# Autodesk Inventor assembly: Chain(d)
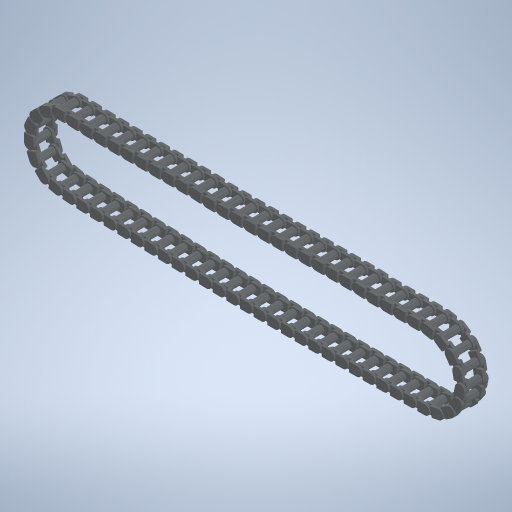
[picture p0: Inventor's stored thumbnail of the model, 512x512]
Saved by Autodesk Inventor 2023 (Build 270158000, 158)
## iProperties
Created: 2022-08-08
Part Number: Chain(d)
Document SubType Name: Assembly
Designer: aaron
Author: aaron
## Documents named in this file (3)
- C:\Users\aaron\Documents\Inventor\Spin Up\library\Motion\New Sprockets\Chain(d).iam
- C:\Users\aaron\Documents\Inventor\Spin Up\library\Motion\New Sprockets\16T.ipt
- C:\Users\aaron\Documents\Inventor\Spin Up\library\Motion\New Sprockets\IQ chain.ipt
## Components (71 placed, 2 different names)
1. 16T:1 — Mate:1, Flush:1, Mate:97, Mate:98, Mate:99, Mate:100, Mate:101, Mate:102, Mate:103, Mate:104, Mate:105
2. 16T:2 — Mate:1, Flush:1, Mate:106, Mate:107, Mate:108, Mate:109, Mate:110, Mate:111, Mate:112, Mate:113, Flush:97
3. IQ chain:6 — Mate:12, Flush:12, Mate:113, Mate:114
4. IQ chain:7 — Mate:12, Flush:12, Mate:112
5. IQ chain:8 — Mate:111
6. IQ chain:9 — Mate:110
7. IQ chain:10 — Mate:109
8. IQ chain:11 — Mate:108
9. IQ chain:12 — Mate:24, Flush:24, Mate:107, Flush:97
10. IQ chain:13 — Mate:24, Flush:24, Mate:106
11. IQ chain:14
12. IQ chain:15
13. IQ chain:16
14. IQ chain:17
15. IQ chain:18
16. IQ chain:19
17. IQ chain:20
18. IQ chain:21
19. IQ chain:22
20. IQ chain:23
21. IQ chain:24 — Mate:48, Flush:48
22. IQ chain:25 — Mate:48, Flush:48
23. IQ chain:26
24. IQ chain:27
25. IQ chain:28
26. IQ chain:29
27. IQ chain:30
28. IQ chain:31
29. IQ chain:32
30. IQ chain:33
31. IQ chain:34
32. IQ chain:35
33. IQ chain:36
34. IQ chain:37
35. IQ chain:38
36. IQ chain:39 — Mate:97
37. IQ chain:40 — Mate:98
38. IQ chain:41 — Mate:99
39. IQ chain:42 — Mate:100
40. IQ chain:43 — Mate:101
41. IQ chain:44 — Mate:102
42. IQ chain:45 — Mate:103
43. IQ chain:46 — Mate:104
44. IQ chain:47 — Mate:105
45. IQ chain:48 — Mate:96, Flush:96
46. IQ chain:49 — Mate:96, Flush:96
47. IQ chain:50
48. IQ chain:51
49. IQ chain:52
50. IQ chain:53
51. IQ chain:54
52. IQ chain:55
53. IQ chain:56
54. IQ chain:57
55. IQ chain:58
56. IQ chain:59
57. IQ chain:60
58. IQ chain:61
59. IQ chain:62
60. IQ chain:63
61. IQ chain:64
62. IQ chain:65
63. IQ chain:66
64. IQ chain:67
65. IQ chain:68
66. IQ chain:69
67. IQ chain:70
68. IQ chain:71
69. IQ chain:72
70. IQ chain:73
71. IQ chain:74 — Mate:114
## Relationships (157: Mate 87, Flush 70)
- Mate:1 (168.402 mm): 16T:1 ↔ 16T:2
- Flush:1: 16T:1 ↔ 16T:2
- [Mate]: IQ chain:7 ↔ IQ chain:8
- [Mate]: IQ chain:8 ↔ IQ chain:9
- [Flush]: IQ chain:7 ↔ IQ chain:8
- [Flush]: IQ chain:8 ↔ IQ chain:9
- [Mate]: IQ chain:10 ↔ IQ chain:11
- [Mate]: IQ chain:11 ↔ IQ chain:12
- [Flush]: IQ chain:10 ↔ IQ chain:11
- [Flush]: IQ chain:11 ↔ IQ chain:12
- [Mate]: IQ chain:9 ↔ IQ chain:10
- [Flush]: IQ chain:9 ↔ IQ chain:10
- Mate:12: IQ chain:6 ↔ IQ chain:7
- Flush:12: IQ chain:6 ↔ IQ chain:7
- [Mate]: IQ chain:13 ↔ IQ chain:14
- [Mate]: IQ chain:14 ↔ IQ chain:15
- [Flush]: IQ chain:13 ↔ IQ chain:14
- [Flush]: IQ chain:14 ↔ IQ chain:15
- [Mate]: IQ chain:16 ↔ IQ chain:17
- [Mate]: IQ chain:17 ↔ IQ chain:18
- [Flush]: IQ chain:16 ↔ IQ chain:17
- [Flush]: IQ chain:17 ↔ IQ chain:18
- [Mate]: IQ chain:15 ↔ IQ chain:16
- [Flush]: IQ chain:15 ↔ IQ chain:16
- [Mate]: IQ chain:19 ↔ IQ chain:20
- [Mate]: IQ chain:20 ↔ IQ chain:21
- [Flush]: IQ chain:19 ↔ IQ chain:20
- [Flush]: IQ chain:20 ↔ IQ chain:21
- [Mate]: IQ chain:22 ↔ IQ chain:23
- [Mate]: IQ chain:23 ↔ IQ chain:24
- [Flush]: IQ chain:22 ↔ IQ chain:23
- [Flush]: IQ chain:23 ↔ IQ chain:24
- [Mate]: IQ chain:21 ↔ IQ chain:22
- [Flush]: IQ chain:21 ↔ IQ chain:22
- [Mate]: IQ chain:18 ↔ IQ chain:19
- [Flush]: IQ chain:18 ↔ IQ chain:19
- Mate:24: IQ chain:12 ↔ IQ chain:13
- Flush:24: IQ chain:12 ↔ IQ chain:13
- [Mate]: IQ chain:25 ↔ IQ chain:26
- [Mate]: IQ chain:26 ↔ IQ chain:27
- [Flush]: IQ chain:25 ↔ IQ chain:26
- [Flush]: IQ chain:26 ↔ IQ chain:27
- [Mate]: IQ chain:28 ↔ IQ chain:29
- [Mate]: IQ chain:29 ↔ IQ chain:30
- [Flush]: IQ chain:28 ↔ IQ chain:29
- [Flush]: IQ chain:29 ↔ IQ chain:30
- [Mate]: IQ chain:27 ↔ IQ chain:28
- [Flush]: IQ chain:27 ↔ IQ chain:28
- [Mate]: IQ chain:31 ↔ IQ chain:32
- [Mate]: IQ chain:32 ↔ IQ chain:33
- [Flush]: IQ chain:31 ↔ IQ chain:32
- [Flush]: IQ chain:32 ↔ IQ chain:33
- [Mate]: IQ chain:34 ↔ IQ chain:35
- [Mate]: IQ chain:35 ↔ IQ chain:36
- [Flush]: IQ chain:34 ↔ IQ chain:35
- [Flush]: IQ chain:35 ↔ IQ chain:36
- [Mate]: IQ chain:33 ↔ IQ chain:34
- [Flush]: IQ chain:33 ↔ IQ chain:34
- [Mate]: IQ chain:30 ↔ IQ chain:31
- [Flush]: IQ chain:30 ↔ IQ chain:31
- [Mate]: IQ chain:37 ↔ IQ chain:38
- [Mate]: IQ chain:38 ↔ IQ chain:39
- [Flush]: IQ chain:37 ↔ IQ chain:38
- [Flush]: IQ chain:38 ↔ IQ chain:39
- [Mate]: IQ chain:40 ↔ IQ chain:41
- [Mate]: IQ chain:41 ↔ IQ chain:42
- [Flush]: IQ chain:40 ↔ IQ chain:41
- [Flush]: IQ chain:41 ↔ IQ chain:42
- [Mate]: IQ chain:39 ↔ IQ chain:40
- [Flush]: IQ chain:39 ↔ IQ chain:40
- [Mate]: IQ chain:43 ↔ IQ chain:44
- [Mate]: IQ chain:44 ↔ IQ chain:45
- [Flush]: IQ chain:43 ↔ IQ chain:44
- [Flush]: IQ chain:44 ↔ IQ chain:45
- [Mate]: IQ chain:46 ↔ IQ chain:47
- [Mate]: IQ chain:47 ↔ IQ chain:48
- [Flush]: IQ chain:46 ↔ IQ chain:47
- [Flush]: IQ chain:47 ↔ IQ chain:48
- [Mate]: IQ chain:45 ↔ IQ chain:46
- [Flush]: IQ chain:45 ↔ IQ chain:46
- [Mate]: IQ chain:42 ↔ IQ chain:43
- [Flush]: IQ chain:42 ↔ IQ chain:43
- [Mate]: IQ chain:36 ↔ IQ chain:37
- [Flush]: IQ chain:36 ↔ IQ chain:37
- Mate:48: IQ chain:24 ↔ IQ chain:25
- Flush:48: IQ chain:24 ↔ IQ chain:25
- [Mate]: IQ chain:49 ↔ IQ chain:50
- [Mate]: IQ chain:50 ↔ IQ chain:51
- [Flush]: IQ chain:49 ↔ IQ chain:50
- [Flush]: IQ chain:50 ↔ IQ chain:51
- [Mate]: IQ chain:52 ↔ IQ chain:53
- [Mate]: IQ chain:53 ↔ IQ chain:54
- [Flush]: IQ chain:52 ↔ IQ chain:53
- [Flush]: IQ chain:53 ↔ IQ chain:54
- [Mate]: IQ chain:51 ↔ IQ chain:52
- [Flush]: IQ chain:51 ↔ IQ chain:52
- [Mate]: IQ chain:55 ↔ IQ chain:56
- [Mate]: IQ chain:56 ↔ IQ chain:57
- [Flush]: IQ chain:55 ↔ IQ chain:56
- [Flush]: IQ chain:56 ↔ IQ chain:57
- [Mate]: IQ chain:58 ↔ IQ chain:59
- [Mate]: IQ chain:59 ↔ IQ chain:60
- [Flush]: IQ chain:58 ↔ IQ chain:59
- [Flush]: IQ chain:59 ↔ IQ chain:60
- [Mate]: IQ chain:57 ↔ IQ chain:58
- [Flush]: IQ chain:57 ↔ IQ chain:58
- [Mate]: IQ chain:54 ↔ IQ chain:55
- [Flush]: IQ chain:54 ↔ IQ chain:55
- [Mate]: IQ chain:61 ↔ IQ chain:62
- [Mate]: IQ chain:62 ↔ IQ chain:63
- [Flush]: IQ chain:61 ↔ IQ chain:62
- [Flush]: IQ chain:62 ↔ IQ chain:63
- [Mate]: IQ chain:64 ↔ IQ chain:65
- [Mate]: IQ chain:65 ↔ IQ chain:66
- [Flush]: IQ chain:64 ↔ IQ chain:65
- [Flush]: IQ chain:65 ↔ IQ chain:66
- [Mate]: IQ chain:63 ↔ IQ chain:64
- [Flush]: IQ chain:63 ↔ IQ chain:64
- [Mate]: IQ chain:67 ↔ IQ chain:68
- [Mate]: IQ chain:68 ↔ IQ chain:69
- [Flush]: IQ chain:67 ↔ IQ chain:68
- [Flush]: IQ chain:68 ↔ IQ chain:69
- [Mate]: IQ chain:70 ↔ IQ chain:71
- [Mate]: IQ chain:71 ↔ IQ chain:72
- [Flush]: IQ chain:70 ↔ IQ chain:71
- [Flush]: IQ chain:71 ↔ IQ chain:72
- [Mate]: IQ chain:69 ↔ IQ chain:70
- [Flush]: IQ chain:69 ↔ IQ chain:70
- [Mate]: IQ chain:66 ↔ IQ chain:67
- [Flush]: IQ chain:66 ↔ IQ chain:67
- [Mate]: IQ chain:60 ↔ IQ chain:61
- [Flush]: IQ chain:60 ↔ IQ chain:61
- [Mate]: IQ chain:73 ↔ IQ chain:74
- [Flush]: IQ chain:73 ↔ IQ chain:74
- [Mate]: IQ chain:72 ↔ IQ chain:73
- [Flush]: IQ chain:72 ↔ IQ chain:73
- Mate:96: IQ chain:48 ↔ IQ chain:49
- Flush:96: IQ chain:48 ↔ IQ chain:49
- Mate:97: 16T:1 ↔ IQ chain:39
- Mate:98: 16T:1 ↔ IQ chain:40
- Mate:99: 16T:1 ↔ IQ chain:41
- Mate:100: 16T:1 ↔ IQ chain:42
- Mate:101: 16T:1 ↔ IQ chain:43
- Mate:102: 16T:1 ↔ IQ chain:44
- Mate:103: 16T:1 ↔ IQ chain:45
- Mate:104: 16T:1 ↔ IQ chain:46
- Mate:105: 16T:1 ↔ IQ chain:47
- Mate:106: 16T:2 ↔ IQ chain:13
- Mate:107: 16T:2 ↔ IQ chain:12
- Mate:108: 16T:2 ↔ IQ chain:11
- Mate:109: 16T:2 ↔ IQ chain:10
- Mate:110: 16T:2 ↔ IQ chain:9
- Mate:111: 16T:2 ↔ IQ chain:8
- Mate:112: 16T:2 ↔ IQ chain:7
- Mate:113: 16T:2 ↔ IQ chain:6
- Mate:114: IQ chain:6 ↔ IQ chain:74
- Flush:97 (-0.762 mm): 16T:2 ↔ IQ chain:12
## Named parameters: d12_d2 = 0 mm, d13_d3 = 0 mm, d14_d4 = 0 mm, d15_d5 = 0 mm, d16_d6_d2 = 0 mm, d17_d7_d3 = 0 mm, d18_d8_d4 = 0 mm, d19_d9_d5 = 0 mm, d20_d10 = 0 mm, d21_d11 = 0 mm, d24_d2 = 0 mm, d25_d3 = 0 mm, d26_d4 = 0 mm, d27_d5 = 0 mm, d28_d6_d2 = 0 mm, d29_d7_d3 = 0 mm, d30_d8_d4 = 0 mm, d31_d9_d5 = 0 mm, d32_d10 = 0 mm, d33_d11 = 0 mm, d34_d12_d2 = 0 mm, d35_d13_d3 = 0 mm, d36_d14_d4 = 0 mm, d37_d15_d5 = 0 mm, d38_d16_d6_d2 = 0 mm, d39_d17_d7_d3 = 0 mm, d40_d18_d8_d4 = 0 mm, d41_d19_d9_d5 = 0 mm, d42_d20_d10 = 0 mm, d43_d21_d11 = 0 mm, d44_d22 = 0 mm, d45_d23 = 0 mm, d48_d2 = 0 mm, d49_d3 = 0 mm, d50_d4 = 0 mm, d51_d5 = 0 mm, d52_d6_d2 = 0 mm, d53_d7_d3 = 0 mm, d54_d8_d4 = 0 mm, d55_d9_d5 = 0 mm, d56_d10 = 0 mm, d57_d11 = 0 mm, d58_d12_d2 = 0 mm, d59_d13_d3 = 0 mm, d60_d14_d4 = 0 mm, d61_d15_d5 = 0 mm, d62_d16_d6_d2 = 0 mm, d63_d17_d7_d3 = 0 mm, d64_d18_d8_d4 = 0 mm, d65_d19_d9_d5 = 0 mm, d66_d20_d10 = 0 mm, d67_d21_d11 = 0 mm, d68_d22 = 0 mm, d69_d23 = 0 mm, d70_d24_d2 = 0 mm, d71_d25_d3 = 0 mm, d72_d26_d4 = 0 mm, d73_d27_d5 = 0 mm, d74_d28_d6_d2 = 0 mm, d75_d29_d7_d3 = 0 mm, d76_d30_d8_d4 = 0 mm, d77_d31_d9_d5 = 0 mm, d78_d32_d10 = 0 mm, d79_d33_d11 = 0 mm, d80_d34_d12_d2 = 0 mm, d81_d35_d13_d3 = 0 mm, d82_d36_d14_d4 = 0 mm, d83_d37_d15_d5 = 0 mm, d84_d38_d16_d6_d2 = 0 mm, d85_d39_d17_d7_d3 = 0 mm, d86_d40_d18_d8_d4 = 0 mm, d87_d41_d19_d9_d5 = 0 mm, d88_d42_d20_d10 = 0 mm, d89_d43_d21_d11 = 0 mm, d90_d44_d22 = 0 mm, d91_d45_d23 = 0 mm, d92_d46 = 0 mm, d93_d47 = 0 mm, d96_d2 = 0 mm, d97_d3 = 0 mm, d98_d4 = 0 mm, d99_d5 = 0 mm, d100_d6_d2 = 0 mm, d101_d7_d3 = 0 mm, d102_d8_d4 = 0 mm, d103_d9_d5 = 0 mm, d104_d10 = 0 mm, d105_d11 = 0 mm, d106_d12_d2 = 0 mm, d107_d13_d3 = 0 mm, d108_d14_d4 = 0 mm, d109_d15_d5 = 0 mm, d110_d16_d6_d2 = 0 mm, d111_d17_d7_d3 = 0 mm, d112_d18_d8_d4 = 0 mm, d113_d19_d9_d5 = 0 mm, d114_d20_d10 = 0 mm, d115_d21_d11 = 0 mm, d116_d22 = 0 mm, d117_d23 = 0 mm, d118_d24_d2 = 0 mm, d119_d25_d3 = 0 mm, d120_d26_d4 = 0 mm, d121_d27_d5 = 0 mm, d122_d28_d6_d2 = 0 mm, d123_d29_d7_d3 = 0 mm, d124_d30_d8_d4 = 0 mm, d125_d31_d9_d5 = 0 mm, d126_d32_d10 = 0 mm, d127_d33_d11 = 0 mm, d128_d34_d12_d2 = 0 mm, d129_d35_d13_d3 = 0 mm, d130_d36_d14_d4 = 0 mm, d131_d37_d15_d5 = 0 mm, d132_d38_d16_d6_d2 = 0 mm, d133_d39_d17_d7_d3 = 0 mm, d134_d40_d18_d8_d4 = 0 mm, d135_d41_d19_d9_d5 = 0 mm, d136_d42_d20_d10 = 0 mm, d137_d43_d21_d11 = 0 mm, d138_d44_d22 = 0 mm, d139_d45_d23 = 0 mm, d140_d94 = 0 mm, d141_d95 = 0 mm, d142_d46 = 0 mm, d143_d47 = 0 mm, d144_d48_d2 = 0 mm, d146_d50_d4 = 0 mm
